# Autodesk Inventor assembly: ASSY GANTRY 5050
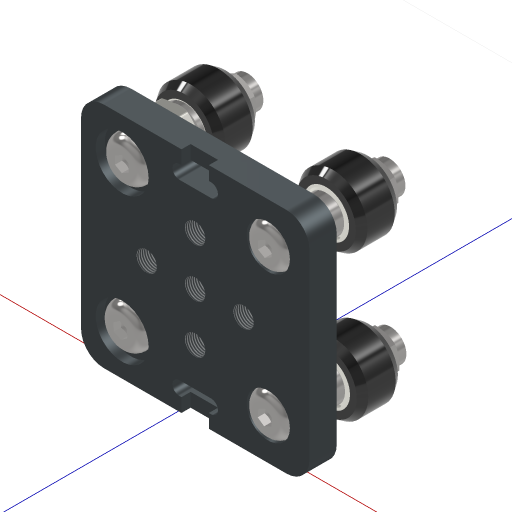
[picture p0: Inventor's stored thumbnail of the model, 512x512]
Saved by Autodesk Inventor 2024.4 (Build 284460000, 460)
## iProperties
Created: 2025-10-22
Part Number: ASSY GANTRY 5050
Document SubType Name: Assembly
Designer: Hp
Author: Hp
## Documents named in this file (8)
- C:\Users\Hp\Pictures\Part TIme Cohexa\Katalog 3D\Gantry 5050\ASSY GANTRY 5050.iam
- C:\Users\Hp\Pictures\Part TIme Cohexa\Katalog 3D\Gantry 5050\Ruber.ipt
- C:\Users\Hp\Documents\Inventor\Content Center Files\R2024\en-US\DIN 985\DIN 985 - M5.ipt
- C:\Users\Hp\Documents\Inventor\Content Center Files\R2024\en-US\ANSI B18.3.4M(2)\ANSI B18.3.4M - M5 x 0.8 x 25(1).ipt
- C:\Users\Hp\Pictures\Part TIme Cohexa\Katalog 3D\Gantry 5050\Washer ID 5 x 7.ipt
- C:\Users\Hp\Pictures\Part TIme Cohexa\Katalog 3D\Gantry 5050\Nuts Gantry.ipt
- C:\Users\Hp\Pictures\Part TIme Cohexa\Katalog 3D\Gantry Base 5050.ipt
- C:\Users\Hp\Documents\Inventor\Content Center Files\R2024\en-US\AS 1237 (2.1)\AS 1237 - 5.ipt
## Components (19 placed, 7 different names)
1. Gantry Base 5050:1 — Mate:3, Rotational:1, Rotational:2, Rotational:14, Rigid:5, Rotational:9, Mate:5, Rotational:10, Mate:7
2. Ruber:1 — Rotational:13, Rotational:12
3. DIN 985 - replaced by DIN EN ISO 10511 M5:1 — Mate:3, Rotational:7
4. Forged Hexagon Socket Button Head Cap Screw - Metric M5 x 0.8 x 25:1 — Mate:6, Mate:7, Mate:10
5. Forged Hexagon Socket Button Head Cap Screw - Metric M5 x 0.8 x 25:2 — Mate:4, Mate:5, Mate:9, Mate:14
6. Forged Hexagon Socket Button Head Cap Screw - Metric M5 x 0.8 x 25:3 — Rotational:1
7. Forged Hexagon Socket Button Head Cap Screw - Metric M5 x 0.8 x 25:4 — Rotational:2
8. Washer ID 5 x 7:1 — Rotational:14, Rotational:13
9. DIN 985 - replaced by DIN EN ISO 10511 M5:2 — Rotational:12
10. Ruber:2 — Rotational:6, Mate:10, Mate:11
11. Ruber:3 — Rotational:8, Rotational:7
12. Ruber:4 — Mate:8, Mate:9, Rotational:11
13. DIN 985 - replaced by DIN EN ISO 10511 M5:3 — Rotational:6
14. DIN 985 - replaced by DIN EN ISO 10511 M5:5 — Rotational:11
15. Washer ID 5 x 7:3 — Rigid:5, Rotational:8
16. Nuts Gantry:3 — Rotational:10, Mate:6, Insert:1
17. Nuts Gantry:4 — Mate:4, Rotational:9, Mate:15
18. AS 1237 (2.1) 5:1 — Mate:14, Mate:15, Mate:8
19. AS 1237 (2.1) 5:2 — Insert:1, Mate:11
## Relationships (24: Mate 11, RevoluteJoint 11, WeldJoint 1, Insert 1)
- Mate:3: Gantry Base 5050:1 ↔ DIN 985 - replaced by DIN EN ISO 10511 M5:1
- Rotational:1 [RevoluteJoint]: Gantry Base 5050:1 ↔ Forged Hexagon Socket Button Head Cap Screw - Metric M5 x 0.8 x 25:3
- Rotational:2 [RevoluteJoint]: Gantry Base 5050:1 ↔ Forged Hexagon Socket Button Head Cap Screw - Metric M5 x 0.8 x 25:4
- Rotational:14 [RevoluteJoint]: Gantry Base 5050:1 ↔ Washer ID 5 x 7:1
- Rotational:13 [RevoluteJoint]: Ruber:1 ↔ Washer ID 5 x 7:1
- Rotational:12 [RevoluteJoint]: Ruber:1 ↔ DIN 985 - replaced by DIN EN ISO 10511 M5:2
- Rotational:6 [RevoluteJoint]: Ruber:2 ↔ DIN 985 - replaced by DIN EN ISO 10511 M5:3
- Rigid:5 [WeldJoint]: Gantry Base 5050:1 ↔ Washer ID 5 x 7:3
- Rotational:8 [RevoluteJoint]: Ruber:3 ↔ Washer ID 5 x 7:3
- Rotational:7 [RevoluteJoint]: DIN 985 - replaced by DIN EN ISO 10511 M5:1 ↔ Ruber:3
- Mate:4: Forged Hexagon Socket Button Head Cap Screw - Metric M5 x 0.8 x 25:2 ↔ Nuts Gantry:4
- Rotational:9 [RevoluteJoint]: Gantry Base 5050:1 ↔ Nuts Gantry:4
- Mate:5: Gantry Base 5050:1 ↔ Forged Hexagon Socket Button Head Cap Screw - Metric M5 x 0.8 x 25:2
- Rotational:10 [RevoluteJoint]: Gantry Base 5050:1 ↔ Nuts Gantry:3
- Mate:6: Forged Hexagon Socket Button Head Cap Screw - Metric M5 x 0.8 x 25:1 ↔ Nuts Gantry:3
- Mate:7: Gantry Base 5050:1 ↔ Forged Hexagon Socket Button Head Cap Screw - Metric M5 x 0.8 x 25:1
- Mate:8: Ruber:4 ↔ AS 1237 (2.1) 5:1
- Mate:9: Forged Hexagon Socket Button Head Cap Screw - Metric M5 x 0.8 x 25:2 ↔ Ruber:4
- Rotational:11 [RevoluteJoint]: Ruber:4 ↔ DIN 985 - replaced by DIN EN ISO 10511 M5:5
- Mate:10: Forged Hexagon Socket Button Head Cap Screw - Metric M5 x 0.8 x 25:1 ↔ Ruber:2
- Mate:11: Ruber:2 ↔ AS 1237 (2.1) 5:2
- Mate:14: Forged Hexagon Socket Button Head Cap Screw - Metric M5 x 0.8 x 25:2 ↔ AS 1237 (2.1) 5:1
- Insert:1: Nuts Gantry:3 ↔ AS 1237 (2.1) 5:2
- Mate:15: Nuts Gantry:4 ↔ AS 1237 (2.1) 5:1
